# Autodesk Inventor assembly: AR-100
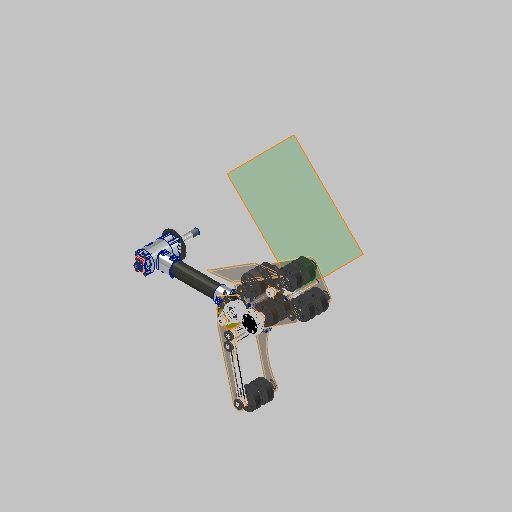
[picture p0: Inventor's stored thumbnail of the model, 512x512]
Saved by Autodesk Inventor 2023.5 (Build 275446000, 446)
## iProperties
Created: 2025-01-22
Part Number: AR-100
Document SubType Name: Assembly
Designer: slick
Mass: 4680.7 g
Surface Area: 11735.1 cm^2
Volume: 2408.47 cm^3
Density: 1.94344 g/cm^3
Author: slick
## Documents named in this file (18)
- C:\Users\slick\OneDrive\Desktop\2025-ReefScape---CAD\Arm\AR-100.iam
- C:\Users\slick\OneDrive\Desktop\2025-ReefScape---CAD\Arm\AR-001.ipt
- C:\Users\slick\OneDrive\Desktop\2025-ReefScape---CAD\COMMON PARTS\BEARINGS\0_875_ID_x_1_875_OD_X_0_500_Radial_Bearing_EE11S-2RS.ipt
- C:\Users\slick\OneDrive\Desktop\2025-ReefScape---CAD\Arm\AR-005.ipt
- C:\Users\slick\OneDrive\Desktop\2025-ReefScape---CAD\Arm\AR-006.ipt
- C:\Users\slick\OneDrive\Desktop\2025-ReefScape---CAD\COMMON PARTS\SPROCKETS\35\WCP-0983\WCP-0983.ipt
- C:\Users\slick\OneDrive\Desktop\2025-ReefScape---CAD\Arm\AR-009.ipt
- C:\Users\slick\OneDrive\Desktop\2025-ReefScape---CAD\Arm\AR-010.ipt
- C:\Users\slick\OneDrive\Desktop\2025-ReefScape---CAD\Gripper\GP3\GP3-100.iam
- C:\Users\slick\OneDrive\Desktop\2025-ReefScape---CAD\Gripper\GP4\GP4-100.iam
- C:\Users\slick\OneDrive\Desktop\2025-ReefScape---CAD\Arm\AR-013.ipt
- C:\Users\slick\OneDrive\Desktop\2025-ReefScape---CAD\Arm\AR-014.ipt
- C:\Users\slick\OneDrive\Desktop\2025-ReefScape---CAD\Elevator\EL2\EL2-A-012.ipt
- C:\Users\slick\OneDrive\Desktop\2025-ReefScape---CAD\Arm\AR-015.ipt
- C:\Users\slick\OneDrive\Desktop\2025-ReefScape---CAD\COMMON PARTS\SDS MK4i Swerve Module, 10-32, Falcons\CANcoder Assembly.iam
- C:\Users\slick\OneDrive\Desktop\2025-ReefScape---CAD\Content Center\en-US\U UNC 2605\Unbrako - 10 x 1 - 24(10).ipt
- C:\Users\slick\OneDrive\Desktop\2025-ReefScape---CAD\Content Center\en-US\U UNC 2605\Unbrako - 10 x 5_16 - 24(10).ipt
- C:\Users\slick\OneDrive\Desktop\2025-ReefScape---CAD\Content Center\en-US\U UNC 2605\Unbrako - 10 x 3_8 - 24(10).ipt
## Components (57 placed, 17 different names)
1. AR-001:1 — Mate:1, Mate:2, Mate:3, Mate:4, Mate:13, Mate:14, Insert:37, Insert:38, Insert:39, Insert:40
2. 0_875_ID_x_1_875_OD_X_0_500_Radial_Bearing_EE11S-2RS:1 — Mate:1, Mate:3, Mate:15, Flush:2, Mate:20
3. 0_875_ID_x_1_875_OD_X_0_500_Radial_Bearing_EE11S-2RS:2 — Mate:2, Mate:4
4. AR-005:1 — Mate:13, Mate:14, Mate:17, Mate:18
5. AR-006:1 — Mate:15, Flush:2, Insert:36, Mate:19, Angle:1
6. WCP-0983:1 — Insert:21, Insert:22, Insert:23, Insert:24, Insert:45, Insert:46, Insert:47, Insert:48
7. AR-009:1 — Insert:21, Insert:22, Insert:23, Insert:24, Insert:39, Insert:40
8. AR-010:1 — Mate:17, Mate:18, Insert:25, Insert:26, Insert:34, Insert:35
9. GP3-100:1 [sub-assembly] — Insert:25, Insert:26
10. GP4-100:1 [sub-assembly] — Insert:34, Insert:35, Angle:1, Insert:57, Insert:58, Insert:59, Insert:60, Insert:61, Insert:62, Insert:63, Insert:64, Insert:65, Insert:66, Insert:67, Insert:68, Insert:69, Insert:70, Insert:71, Insert:72, Insert:73, Insert:74, Insert:75, Insert:76, Insert:77, Insert:78, Insert:82, Insert:83, Insert:84, Insert:85, Insert:86, Insert:87, Insert:91, Insert:92
11. AR-013:1 — Insert:36
12. AR-014:1 — Insert:37, Insert:38, Insert:41, Insert:42, Insert:49, Insert:50, Insert:51, Insert:52
13. EL2-A-012:1 — Mate:19, Mate:20
14. AR-015:1 — Insert:41, Insert:42, Insert:43, Insert:44, Insert:53, Insert:54, Insert:55, Insert:56
15. CANcoder Assembly:1 [sub-assembly] — Insert:43, Insert:44
16. Unbrako UNC Hex Socket Button Cap - Inch 10 x 1:1 — Insert:45
17. Unbrako UNC Hex Socket Button Cap - Inch 10 x 1:2 — Insert:46
18. Unbrako UNC Hex Socket Button Cap - Inch 10 x 1:3 — Insert:47
19. Unbrako UNC Hex Socket Button Cap - Inch 10 x 1:4 — Insert:48
20. Unbrako UNC Hex Socket Button Cap - Inch 10 x 1:5 — Insert:49
21. Unbrako UNC Hex Socket Button Cap - Inch 10 x 1:6 — Insert:50
22. Unbrako UNC Hex Socket Button Cap - Inch 10 x 1:7 — Insert:51
23. Unbrako UNC Hex Socket Button Cap - Inch 10 x 1:8 — Insert:52
24. Unbrako UNC Hex Socket Button Cap - Inch 10 x 5/16:1 — Insert:53
25. Unbrako UNC Hex Socket Button Cap - Inch 10 x 5/16:2 — Insert:54
26. Unbrako UNC Hex Socket Button Cap - Inch 10 x 5/16:3 — Insert:55
27. Unbrako UNC Hex Socket Button Cap - Inch 10 x 5/16:4 — Insert:56
28. Unbrako UNC Hex Socket Button Cap - Inch 10 x 1:9 — Insert:57
29. Unbrako UNC Hex Socket Button Cap - Inch 10 x 1:10 — Insert:58
30. Unbrako UNC Hex Socket Button Cap - Inch 10 x 1:11 — Insert:59
31. Unbrako UNC Hex Socket Button Cap - Inch 10 x 1:12 — Insert:60
32. Unbrako UNC Hex Socket Button Cap - Inch 10 x 3/8:1 — Insert:61
33. Unbrako UNC Hex Socket Button Cap - Inch 10 x 3/8:2 — Insert:62
34. Unbrako UNC Hex Socket Button Cap - Inch 10 x 3/8:3 — Insert:63
35. Unbrako UNC Hex Socket Button Cap - Inch 10 x 3/8:4 — Insert:64
36. Unbrako UNC Hex Socket Button Cap - Inch 10 x 3/8:5 — Insert:65
37. Unbrako UNC Hex Socket Button Cap - Inch 10 x 3/8:6 — Insert:66
38. Unbrako UNC Hex Socket Button Cap - Inch 10 x 3/8:7 — Insert:67
39. Unbrako UNC Hex Socket Button Cap - Inch 10 x 3/8:8 — Insert:68
40. Unbrako UNC Hex Socket Button Cap - Inch 10 x 3/8:9 — Insert:69
41. Unbrako UNC Hex Socket Button Cap - Inch 10 x 3/8:10 — Insert:70
42. Unbrako UNC Hex Socket Button Cap - Inch 10 x 3/8:11 — Insert:71
43. Unbrako UNC Hex Socket Button Cap - Inch 10 x 3/8:12 — Insert:72
44. Unbrako UNC Hex Socket Button Cap - Inch 10 x 3/8:13 — Insert:73
45. Unbrako UNC Hex Socket Button Cap - Inch 10 x 3/8:14 — Insert:74
46. Unbrako UNC Hex Socket Button Cap - Inch 10 x 3/8:15 — Insert:75
47. Unbrako UNC Hex Socket Button Cap - Inch 10 x 3/8:16 — Insert:76
48. Unbrako UNC Hex Socket Button Cap - Inch 10 x 3/8:17 — Insert:77
49. Unbrako UNC Hex Socket Button Cap - Inch 10 x 3/8:18 — Insert:78
50. Unbrako UNC Hex Socket Button Cap - Inch 10 x 3/8:22 — Insert:82
51. Unbrako UNC Hex Socket Button Cap - Inch 10 x 3/8:23 — Insert:83
52. Unbrako UNC Hex Socket Button Cap - Inch 10 x 3/8:24 — Insert:84
53. Unbrako UNC Hex Socket Button Cap - Inch 10 x 3/8:25 — Insert:85
54. Unbrako UNC Hex Socket Button Cap - Inch 10 x 3/8:26 — Insert:86
55. Unbrako UNC Hex Socket Button Cap - Inch 10 x 3/8:27 — Insert:87
56. Unbrako UNC Hex Socket Button Cap - Inch 10 x 3/8:31 — Insert:91
57. Unbrako UNC Hex Socket Button Cap - Inch 10 x 3/8:32 — Insert:92
## Relationships (72: Insert 59, Mate 11, Flush 1, Angle 1)
- Mate:1: AR-001:1 ↔ 0_875_ID_x_1_875_OD_X_0_500_Radial_Bearing_EE11S-2RS:1
- Mate:2: AR-001:1 ↔ 0_875_ID_x_1_875_OD_X_0_500_Radial_Bearing_EE11S-2RS:2
- Mate:3: AR-001:1 ↔ 0_875_ID_x_1_875_OD_X_0_500_Radial_Bearing_EE11S-2RS:1
- Mate:4: AR-001:1 ↔ 0_875_ID_x_1_875_OD_X_0_500_Radial_Bearing_EE11S-2RS:2
- Mate:13: AR-001:1 ↔ AR-005:1
- Mate:14 (-50.8 mm): AR-001:1 ↔ AR-005:1
- Mate:15: 0_875_ID_x_1_875_OD_X_0_500_Radial_Bearing_EE11S-2RS:1 ↔ AR-006:1
- Flush:2 (-12.7 mm): 0_875_ID_x_1_875_OD_X_0_500_Radial_Bearing_EE11S-2RS:1 ↔ AR-006:1
- Insert:21: WCP-0983:1 ↔ AR-009:1
- Insert:22: WCP-0983:1 ↔ AR-009:1
- Insert:23: WCP-0983:1 ↔ AR-009:1
- Insert:24: WCP-0983:1 ↔ AR-009:1
- Mate:17: AR-005:1 ↔ AR-010:1
- Mate:18: AR-005:1 ↔ AR-010:1
- Insert:25: AR-010:1 ↔ GP3-100:1
- Insert:26: AR-010:1 ↔ GP3-100:1
- Insert:34: AR-010:1 ↔ GP4-100:1
- Insert:35: AR-010:1 ↔ GP4-100:1
- Insert:36: AR-006:1 ↔ AR-013:1
- Insert:37: AR-001:1 ↔ AR-014:1
- Insert:38: AR-001:1 ↔ AR-014:1
- Insert:39: AR-001:1 ↔ AR-009:1
- Insert:40: AR-001:1 ↔ AR-009:1
- Mate:19: AR-006:1 ↔ EL2-A-012:1
- Mate:20: 0_875_ID_x_1_875_OD_X_0_500_Radial_Bearing_EE11S-2RS:1 ↔ EL2-A-012:1
- Insert:41: AR-014:1 ↔ AR-015:1
- Insert:42: AR-014:1 ↔ AR-015:1
- Insert:43: AR-015:1 ↔ CANcoder Assembly:1
- Insert:44: AR-015:1 ↔ CANcoder Assembly:1
- Angle:1 (0 deg): AR-006:1 ↔ GP4-100:1
- Insert:45: WCP-0983:1 ↔ Unbrako UNC Hex Socket Button Cap - Inch 10 x 1:1
- Insert:46: WCP-0983:1 ↔ Unbrako UNC Hex Socket Button Cap - Inch 10 x 1:2
- Insert:47: WCP-0983:1 ↔ Unbrako UNC Hex Socket Button Cap - Inch 10 x 1:3
- Insert:48: WCP-0983:1 ↔ Unbrako UNC Hex Socket Button Cap - Inch 10 x 1:4
- Insert:49: AR-014:1 ↔ Unbrako UNC Hex Socket Button Cap - Inch 10 x 1:5
- Insert:50: AR-014:1 ↔ Unbrako UNC Hex Socket Button Cap - Inch 10 x 1:6
- Insert:51: AR-014:1 ↔ Unbrako UNC Hex Socket Button Cap - Inch 10 x 1:7
- Insert:52: AR-014:1 ↔ Unbrako UNC Hex Socket Button Cap - Inch 10 x 1:8
- Insert:53: AR-015:1 ↔ Unbrako UNC Hex Socket Button Cap - Inch 10 x 5/16:1
- Insert:54: AR-015:1 ↔ Unbrako UNC Hex Socket Button Cap - Inch 10 x 5/16:2
- Insert:55: AR-015:1 ↔ Unbrako UNC Hex Socket Button Cap - Inch 10 x 5/16:3
- Insert:56: AR-015:1 ↔ Unbrako UNC Hex Socket Button Cap - Inch 10 x 5/16:4
- Insert:57: GP4-100:1 ↔ Unbrako UNC Hex Socket Button Cap - Inch 10 x 1:9
- Insert:58: GP4-100:1 ↔ Unbrako UNC Hex Socket Button Cap - Inch 10 x 1:10
- Insert:59: GP4-100:1 ↔ Unbrako UNC Hex Socket Button Cap - Inch 10 x 1:11
- Insert:60: GP4-100:1 ↔ Unbrako UNC Hex Socket Button Cap - Inch 10 x 1:12
- Insert:61: GP4-100:1 ↔ Unbrako UNC Hex Socket Button Cap - Inch 10 x 3/8:1
- Insert:62: GP4-100:1 ↔ Unbrako UNC Hex Socket Button Cap - Inch 10 x 3/8:2
- Insert:63: GP4-100:1 ↔ Unbrako UNC Hex Socket Button Cap - Inch 10 x 3/8:3
- Insert:64: GP4-100:1 ↔ Unbrako UNC Hex Socket Button Cap - Inch 10 x 3/8:4
- Insert:65: GP4-100:1 ↔ Unbrako UNC Hex Socket Button Cap - Inch 10 x 3/8:5
- Insert:66: GP4-100:1 ↔ Unbrako UNC Hex Socket Button Cap - Inch 10 x 3/8:6
- Insert:67: GP4-100:1 ↔ Unbrako UNC Hex Socket Button Cap - Inch 10 x 3/8:7
- Insert:68: GP4-100:1 ↔ Unbrako UNC Hex Socket Button Cap - Inch 10 x 3/8:8
- Insert:69: GP4-100:1 ↔ Unbrako UNC Hex Socket Button Cap - Inch 10 x 3/8:9
- Insert:70: GP4-100:1 ↔ Unbrako UNC Hex Socket Button Cap - Inch 10 x 3/8:10
- Insert:71: GP4-100:1 ↔ Unbrako UNC Hex Socket Button Cap - Inch 10 x 3/8:11
- Insert:72: GP4-100:1 ↔ Unbrako UNC Hex Socket Button Cap - Inch 10 x 3/8:12
- Insert:73: GP4-100:1 ↔ Unbrako UNC Hex Socket Button Cap - Inch 10 x 3/8:13
- Insert:74: GP4-100:1 ↔ Unbrako UNC Hex Socket Button Cap - Inch 10 x 3/8:14
- Insert:75: GP4-100:1 ↔ Unbrako UNC Hex Socket Button Cap - Inch 10 x 3/8:15
- Insert:76: GP4-100:1 ↔ Unbrako UNC Hex Socket Button Cap - Inch 10 x 3/8:16
- Insert:77: GP4-100:1 ↔ Unbrako UNC Hex Socket Button Cap - Inch 10 x 3/8:17
- Insert:78: GP4-100:1 ↔ Unbrako UNC Hex Socket Button Cap - Inch 10 x 3/8:18
- Insert:82: GP4-100:1 ↔ Unbrako UNC Hex Socket Button Cap - Inch 10 x 3/8:22
- Insert:83: GP4-100:1 ↔ Unbrako UNC Hex Socket Button Cap - Inch 10 x 3/8:23
- Insert:84: GP4-100:1 ↔ Unbrako UNC Hex Socket Button Cap - Inch 10 x 3/8:24
- Insert:85: GP4-100:1 ↔ Unbrako UNC Hex Socket Button Cap - Inch 10 x 3/8:25
- Insert:86: GP4-100:1 ↔ Unbrako UNC Hex Socket Button Cap - Inch 10 x 3/8:26
- Insert:87: GP4-100:1 ↔ Unbrako UNC Hex Socket Button Cap - Inch 10 x 3/8:27
- Insert:91: GP4-100:1 ↔ Unbrako UNC Hex Socket Button Cap - Inch 10 x 3/8:31
- Insert:92: GP4-100:1 ↔ Unbrako UNC Hex Socket Button Cap - Inch 10 x 3/8:32
